# Autodesk Inventor assembly: FullBoard
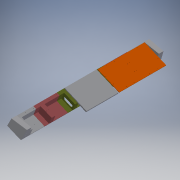
[picture p0: Inventor's stored thumbnail of the model, 180x180]
Saved by Autodesk Inventor 2019 (Build 230136000, 136)
## iProperties
Created: 2019-01-04
Part Number: FullBoard
Document SubType Name: Assembly
Designer: james
Author: james
## Documents named in this file (9)
- F:\JimsDesign\4089DriversStation\FullBoard.iam
- F:\JimsDesign\4089DriversStation\ControlPlate.ipt
- F:\JimsDesign\4089DriversStation\CPLRightOne.ipt
- F:\JimsDesign\4089DriversStation\CPLRightTwo.ipt
- F:\JimsDesign\4089DriversStation\CPLRightThree.ipt
- F:\JimsDesign\4089DriversStation\CPLLeftThree.ipt
- F:\JimsDesign\4089DriversStation\CPLLeftTwo.ipt
- F:\JimsDesign\4089DriversStation\CPLLeftOne.ipt
- F:\JimsDesign\4089DriversStation\SurfaceBook2.ipt
## Components (9 placed, 8 different names)
1. ControlPlate:1 — Mate:5, Mate:8, Flush:4, Mate:13
2. CPLRightOne:1 — Mate:5, Mate:6, Flush:2, Flush:3
3. CPLRightTwo:1 — Mate:6, Flush:2, Flush:3, Mate:7, Mate:9, Flush:5, Flush:6
4. ControlPlate:2 — Mate:7, Mate:8, Flush:4
5. CPLRightThree:1 — Mate:9, Flush:5, Flush:6, Mate:10, Flush:7, Flush:8
6. CPLLeftThree:1 — Mate:10, Flush:7, Flush:8, Mate:11, Flush:9, Flush:10, Mate:14
7. CPLLeftTwo:1 — Mate:11, Flush:9, Flush:10, Mate:12, Flush:11, Flush:12
8. CPLLeftOne:1 — Mate:12, Flush:11, Flush:12, Mate:13
9. SurfaceBook2:1 — Mate:14
## Relationships (21: Flush 11, Mate 10)
- Mate:5: ControlPlate:1 ↔ CPLRightOne:1
- Mate:6: CPLRightOne:1 ↔ CPLRightTwo:1
- Flush:2: CPLRightOne:1 ↔ CPLRightTwo:1
- Flush:3: CPLRightOne:1 ↔ CPLRightTwo:1
- Mate:7: CPLRightTwo:1 ↔ ControlPlate:2
- Mate:8: ControlPlate:1 ↔ ControlPlate:2
- Flush:4: ControlPlate:1 ↔ ControlPlate:2
- Mate:9: CPLRightTwo:1 ↔ CPLRightThree:1
- Flush:5: CPLRightTwo:1 ↔ CPLRightThree:1
- Flush:6: CPLRightTwo:1 ↔ CPLRightThree:1
- Mate:10: CPLRightThree:1 ↔ CPLLeftThree:1
- Flush:7: CPLRightThree:1 ↔ CPLLeftThree:1
- Flush:8: CPLRightThree:1 ↔ CPLLeftThree:1
- Mate:11: CPLLeftThree:1 ↔ CPLLeftTwo:1
- Flush:9: CPLLeftThree:1 ↔ CPLLeftTwo:1
- Flush:10: CPLLeftThree:1 ↔ CPLLeftTwo:1
- Mate:12: CPLLeftTwo:1 ↔ CPLLeftOne:1
- Flush:11: CPLLeftTwo:1 ↔ CPLLeftOne:1
- Flush:12: CPLLeftTwo:1 ↔ CPLLeftOne:1
- Mate:13: ControlPlate:1 ↔ CPLLeftOne:1
- Mate:14: CPLLeftThree:1 ↔ SurfaceBook2:1
